# Autodesk Inventor assembly: Pont+Motor
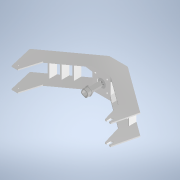
[picture p0: Inventor's stored thumbnail of the model, 180x180]
Saved by Autodesk Inventor 2021 (Build 250183000, 183)
## iProperties
Created: 2021-04-15
Part Number: Pont+Motor
Document SubType Name: Assembly
Designer: Marc
Author: Marc
## Documents named in this file (4)
- C:\Users\Marc\Documents\Projectes\Rubik's Cube Solver\Prototip Definitiu\Pont+Motor.iam
- C:\Users\Marc\Documents\Projectes\Rubik's Cube Solver\Prototip Definitiu\Components\Pont Motor Definitiu.ipt
- C:\Users\Marc\Documents\Projectes\Rubik's Cube Solver\Prototip Definitiu\Components\Nema17\Steppermotor 17HS4417 1.7A 1.8° 2.55V v6_TOP.iam
- C:\Users\Marc\Documents\Projectes\Rubik's Cube Solver\Prototip Definitiu\Components\Eix Superior i Inferior.ipt
## Components (3 placed, 3 different names)
1. Pont Motor Definitiu:1 — Coincidencia:1, Coincidencia:2, Coincidencia:3
2. Steppermotor 17HS4417 1.7A 1.8° 2.55V v6_TOP:1 [sub-assembly] — Coincidencia:1, Coincidencia:2, Coincidencia:3, Coincidencia:4, Coincidencia:5
3. Eix Superior i Inferior:1 — Coincidencia:4, Coincidencia:5
## Relationships (5: Mate 5)
- Coincidencia:1 [Mate]: Pont Motor Definitiu:1 ↔ Steppermotor 17HS4417 1.7A 1.8° 2.55V v6_TOP:1
- Coincidencia:2 [Mate]: Pont Motor Definitiu:1 ↔ Steppermotor 17HS4417 1.7A 1.8° 2.55V v6_TOP:1
- Coincidencia:3 [Mate]: Pont Motor Definitiu:1 ↔ Steppermotor 17HS4417 1.7A 1.8° 2.55V v6_TOP:1
- Coincidencia:4 [Mate]: Steppermotor 17HS4417 1.7A 1.8° 2.55V v6_TOP:1 ↔ Eix Superior i Inferior:1
- Coincidencia:5 [Mate]: Steppermotor 17HS4417 1.7A 1.8° 2.55V v6_TOP:1 ↔ Eix Superior i Inferior:1
